# Autodesk Inventor assembly: ensamble
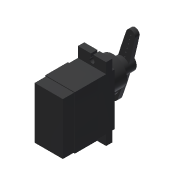
[picture p0: Inventor's stored thumbnail of the model, 180x180]
Saved by Autodesk Inventor 2016 (Build 200138000, 138)
## iProperties
Created: 2016-07-30
Part Number: ensamble
Document SubType Name: Assembly
Designer: julianesteban
Author: julianesteban
## Documents named in this file (5)
- C:\Users\julianesteban\Documents\MEGA\Julián y Espitia\diseños inventor elementos comerciales\motores\servo motor MG90S\ensamble.iam
- C:\Users\julianesteban\Documents\MEGA\Julián y Espitia\diseños inventor elementos comerciales\motores\servo motor MG90S\servo 2.ipt
- C:\Users\julianesteban\Documents\MEGA\Julián y Espitia\diseños inventor elementos comerciales\motores\servo motor MG90S\servo.ipt
- C:\Users\julianesteban\Documents\MEGA\Julián y Espitia\diseños inventor elementos comerciales\motores\servo motor MG90S\servo 3.ipt
- C:\Users\julianesteban\Documents\MEGA\Julián y Espitia\diseños inventor elementos comerciales\motores\servo motor MG90S\servo 4.ipt
## Components (4 placed, 4 different names)
1. servo 2:1 — Mate:1, Mate:2, Mate:3, Mate:4
2. servo:1 — Mate:1, Mate:2
3. servo 3:1 — Mate:3, Mate:4, Mate:5, Mate:6, Mate:7
4. servo 4:1 — Mate:5, Mate:6, Mate:7
## Relationships (7: Mate 7)
- Mate:1: servo 2:1 ↔ servo:1
- Mate:2: servo 2:1 ↔ servo:1
- Mate:3: servo 2:1 ↔ servo 3:1
- Mate:4: servo 2:1 ↔ servo 3:1
- Mate:5: servo 3:1 ↔ servo 4:1
- Mate:6: servo 3:1 ↔ servo 4:1
- Mate:7: servo 3:1 ↔ servo 4:1
